# Autodesk Inventor assembly: (FINAL)2SIDEROLLER
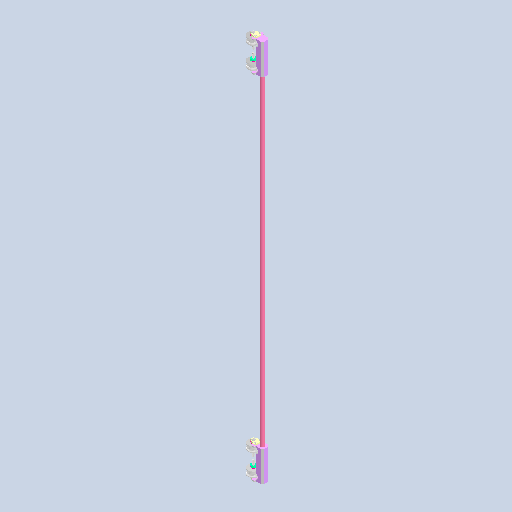
[picture p0: Inventor's stored thumbnail of the model, 512x512]
Saved by Autodesk Inventor 2022 (Build 260153000, 153)
## iProperties
Created: 2022-11-16
Part Number: (FINAL)2SIDEROLLER
Document SubType Name: Assembly
Designer: matia
Author: matia
## Documents named in this file (3)
- C:\Users\matia\Desktop\(V2) FULL ASSEMBLY\(FINAL)2SIDEROLLER.iam
- C:\Users\matia\Desktop\(V2) FULL ASSEMBLY\blockrod.ipt
- C:\Users\matia\Desktop\(V2) FULL ASSEMBLY\(FINAL)rollerAssembly.iam
## Components (3 placed, 2 different names)
1. blockrod:1 — Mate:1, Mate:2, Mate:3, Mate:4
2. (FINAL)rollerAssembly:1 [sub-assembly] — Mate:1, Mate:2
3. (FINAL)rollerAssembly:2 [sub-assembly] — Mate:3, Mate:4
## Relationships (4: Mate 4)
- Mate:1: blockrod:1 ↔ (FINAL)rollerAssembly:1
- Mate:2: blockrod:1 ↔ (FINAL)rollerAssembly:1
- Mate:3: blockrod:1 ↔ (FINAL)rollerAssembly:2
- Mate:4: blockrod:1 ↔ (FINAL)rollerAssembly:2
